# Autodesk Inventor assembly: Assembly12
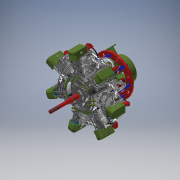
[picture p0: Inventor's stored thumbnail of the model, 180x180]
Saved by Autodesk Inventor 2018 (Build 220112000, 112)
## iProperties
Created: 2023-05-03
Part Number: Assembly12
Document SubType Name: Assembly
Designer: Habib Mohamed
Author: Habib Mohamed
## Documents named in this file (11)
- D:\Inventor\My projects\Rotary Engine\Assembly\Assembly12.iam
- D:\Inventor\My projects\Rotary Engine\Assembly\Assembly10(Suction houe sub assembly).iam
- D:\Inventor\My projects\Rotary Engine\Assembly\Assembly9 (Crank Case Sub Assembly).iam
- D:\Inventor\My projects\Rotary Engine\Component 9 (Suspension Spacer).ipt
- D:\Inventor\My projects\Rotary Engine\Component 10(Assembly Ring).ipt
- D:\Inventor\My projects\Rotary Engine\Assembly\Assembly2 (Intake Pipe Sub Assembly).iam
- C:\Users\Habib Mohamed\Downloads\Exhaust Pipe Sub-Assembly.iam
- D:\Inventor\My projects\Rotary Engine\Component 46(Engine Gas Collector).ipt
- C:\Users\Habib Mohamed\Documents\Inventor\Content Center Files\R2018\en-US\ISO 4762(1)\DIN EN ISO 4762 - M3 x 5.ipt
- C:\Users\Habib Mohamed\Documents\Inventor\Content Center Files\R2018\en-US\ISO 4762(1)\DIN EN ISO 4762 - M4 x 10.ipt
- C:\Users\Habib Mohamed\Documents\Inventor\Content Center Files\R2018\en-US\ISO 10511\ISO 10511 - M5.ipt
## Components (67 placed, 10 different names)
1. Assembly10(Suction houe sub assembly):1 [sub-assembly] — Mate:1, Mate:2, Mate:3, Mate:28, Mate:30, Mate:32, Mate:34, Mate:36, Mate:38, Mate:40
2. Assembly9 (Crank Case Sub Assembly):1 [sub-assembly] — Mate:1, Mate:2, Mate:3, Mate:4, Mate:5, Mate:6, Mate:9, Mate:10, Mate:11, Mate:12, Mate:13, Mate:14, Mate:15, Mate:19, Mate:21, Mate:23, Mate:25, Mate:27, Mate:29, Mate:31, Mate:33, Mate:35, Mate:37, Mate:39
3. Component 10(Assembly Ring):1 — Mate:6, Mate:7, Mate:8, Mate:42
4. Component 46(Engine Gas Collector):1 — Mate:15, Mate:16, Mate:17, Mate:18, Mate:43
5. DIN EN ISO 4762 M4 x 10:1 — Mate:27, Mate:28
6. DIN EN ISO 4762 M4 x 10:2 — Mate:29, Mate:30
7. DIN EN ISO 4762 M4 x 10:3 — Mate:31, Mate:32
8. DIN EN ISO 4762 M4 x 10:4 — Mate:33, Mate:34
9. DIN EN ISO 4762 M4 x 10:5 — Mate:35, Mate:36
10. DIN EN ISO 4762 M4 x 10:6 — Mate:37, Mate:38
11. DIN EN ISO 4762 M4 x 10:7 — Mate:39, Mate:40
12. DIN EN ISO 4762 M3 x 5:1 — Mate:19, Mate:20
13. DIN EN ISO 4762 M3 x 5:2 — Mate:21, Mate:22
14. Assembly2 (Intake Pipe Sub Assembly):1 [sub-assembly] — Mate:9, Mate:10, Mate:11, Mate:20, Mate:22
15. Component 9 (Suspension Spacer):1 — Mate:4, Mate:5, Mate:7, Mate:8, Mate:41
16. DIN EN ISO 10511 M5:1 — Mate:41, Mate:42
17. DIN EN ISO 4762 M3 x 5:3 — Mate:23, Mate:24
18. DIN EN ISO 4762 M3 x 5:4 — Mate:25, Mate:26
19. Exhaust Pipe Sub-Assembly:1 [sub-assembly] — Mate:12, Mate:13, Mate:14, Mate:17, Mate:18, Mate:24, Mate:26
20. DIN EN ISO 4762 M3 x 5:5
21. DIN EN ISO 4762 M3 x 5:6
22. Assembly2 (Intake Pipe Sub Assembly):2 [sub-assembly]
23. Component 9 (Suspension Spacer):2
24. DIN EN ISO 10511 M5:2
25. DIN EN ISO 4762 M3 x 5:7
26. DIN EN ISO 4762 M3 x 5:8
27. Exhaust Pipe Sub-Assembly:2 [sub-assembly]
28. DIN EN ISO 4762 M3 x 5:9
29. DIN EN ISO 4762 M3 x 5:10
30. Assembly2 (Intake Pipe Sub Assembly):3 [sub-assembly]
31. Component 9 (Suspension Spacer):3
32. DIN EN ISO 10511 M5:3
33. DIN EN ISO 4762 M3 x 5:11
34. DIN EN ISO 4762 M3 x 5:12
35. Exhaust Pipe Sub-Assembly:3 [sub-assembly]
36. DIN EN ISO 4762 M3 x 5:13
37. DIN EN ISO 4762 M3 x 5:14
38. Assembly2 (Intake Pipe Sub Assembly):4 [sub-assembly]
39. Component 9 (Suspension Spacer):4
40. DIN EN ISO 10511 M5:4
41. DIN EN ISO 4762 M3 x 5:15
42. DIN EN ISO 4762 M3 x 5:16
43. Exhaust Pipe Sub-Assembly:4 [sub-assembly]
44. DIN EN ISO 4762 M3 x 5:17
45. DIN EN ISO 4762 M3 x 5:18
46. Assembly2 (Intake Pipe Sub Assembly):5 [sub-assembly]
47. Component 9 (Suspension Spacer):5
48. DIN EN ISO 10511 M5:5
49. DIN EN ISO 4762 M3 x 5:19
50. DIN EN ISO 4762 M3 x 5:20
51. Exhaust Pipe Sub-Assembly:5 [sub-assembly]
52. DIN EN ISO 4762 M3 x 5:21
53. DIN EN ISO 4762 M3 x 5:22
54. Assembly2 (Intake Pipe Sub Assembly):6 [sub-assembly]
55. Component 9 (Suspension Spacer):6
56. DIN EN ISO 10511 M5:6
57. DIN EN ISO 4762 M3 x 5:23
58. DIN EN ISO 4762 M3 x 5:24
59. Exhaust Pipe Sub-Assembly:6 [sub-assembly]
60. DIN EN ISO 4762 M3 x 5:25
61. DIN EN ISO 4762 M3 x 5:26
62. Assembly2 (Intake Pipe Sub Assembly):7 [sub-assembly]
63. Component 9 (Suspension Spacer):7
64. DIN EN ISO 10511 M5:7
65. DIN EN ISO 4762 M3 x 5:27
66. DIN EN ISO 4762 M3 x 5:28
67. Exhaust Pipe Sub-Assembly:7 [sub-assembly]
## Component patterns: (7 elements, first: DIN EN ISO 4762 M3 x 5:1 + DIN EN ISO 4762 M3 x 5:2 + Assembly2 (Intake Pipe Sub Assembly):1 + Component 9 (Suspension Spacer):1 + DIN EN ISO 10511 M5:1 + DIN EN ISO 4762 M3 x 5:3 + DIN EN ISO 4762 M3 x 5:4 + Exhaust Pipe Sub-Assembly:1)
## Relationships (43: Mate 43)
- Mate:1: Assembly10(Suction houe sub assembly):1 ↔ Assembly9 (Crank Case Sub Assembly):1
- Mate:2: Assembly10(Suction houe sub assembly):1 ↔ Assembly9 (Crank Case Sub Assembly):1
- Mate:3: Assembly10(Suction houe sub assembly):1 ↔ Assembly9 (Crank Case Sub Assembly):1
- Mate:4: Assembly9 (Crank Case Sub Assembly):1 ↔ Component 9 (Suspension Spacer):1
- Mate:5: Assembly9 (Crank Case Sub Assembly):1 ↔ Component 9 (Suspension Spacer):1
- Mate:6: Assembly9 (Crank Case Sub Assembly):1 ↔ Component 10(Assembly Ring):1
- Mate:7: Component 10(Assembly Ring):1 ↔ Component 9 (Suspension Spacer):1
- Mate:8: Component 10(Assembly Ring):1 ↔ Component 9 (Suspension Spacer):1
- Mate:9: Assembly9 (Crank Case Sub Assembly):1 ↔ Assembly2 (Intake Pipe Sub Assembly):1
- Mate:10: Assembly9 (Crank Case Sub Assembly):1 ↔ Assembly2 (Intake Pipe Sub Assembly):1
- Mate:11: Assembly9 (Crank Case Sub Assembly):1 ↔ Assembly2 (Intake Pipe Sub Assembly):1
- Mate:12: Assembly9 (Crank Case Sub Assembly):1 ↔ Exhaust Pipe Sub-Assembly:1
- Mate:13: Assembly9 (Crank Case Sub Assembly):1 ↔ Exhaust Pipe Sub-Assembly:1
- Mate:14: Assembly9 (Crank Case Sub Assembly):1 ↔ Exhaust Pipe Sub-Assembly:1
- Mate:15: Assembly9 (Crank Case Sub Assembly):1 ↔ Component 46(Engine Gas Collector):1
- Mate:16: Component 46(Engine Gas Collector):1
- Mate:17: Component 46(Engine Gas Collector):1 ↔ Exhaust Pipe Sub-Assembly:1
- Mate:18: Component 46(Engine Gas Collector):1 ↔ Exhaust Pipe Sub-Assembly:1
- Mate:19: Assembly9 (Crank Case Sub Assembly):1 ↔ DIN EN ISO 4762 M3 x 5:1
- Mate:20: DIN EN ISO 4762 M3 x 5:1 ↔ Assembly2 (Intake Pipe Sub Assembly):1
- Mate:21: Assembly9 (Crank Case Sub Assembly):1 ↔ DIN EN ISO 4762 M3 x 5:2
- Mate:22: DIN EN ISO 4762 M3 x 5:2 ↔ Assembly2 (Intake Pipe Sub Assembly):1
- Mate:23: Assembly9 (Crank Case Sub Assembly):1 ↔ DIN EN ISO 4762 M3 x 5:3
- Mate:24: DIN EN ISO 4762 M3 x 5:3 ↔ Exhaust Pipe Sub-Assembly:1
- Mate:25: Assembly9 (Crank Case Sub Assembly):1 ↔ DIN EN ISO 4762 M3 x 5:4
- Mate:26: DIN EN ISO 4762 M3 x 5:4 ↔ Exhaust Pipe Sub-Assembly:1
- Mate:27: Assembly9 (Crank Case Sub Assembly):1 ↔ DIN EN ISO 4762 M4 x 10:1
- Mate:28: Assembly10(Suction houe sub assembly):1 ↔ DIN EN ISO 4762 M4 x 10:1
- Mate:29: Assembly9 (Crank Case Sub Assembly):1 ↔ DIN EN ISO 4762 M4 x 10:2
- Mate:30: Assembly10(Suction houe sub assembly):1 ↔ DIN EN ISO 4762 M4 x 10:2
- Mate:31: Assembly9 (Crank Case Sub Assembly):1 ↔ DIN EN ISO 4762 M4 x 10:3
- Mate:32: Assembly10(Suction houe sub assembly):1 ↔ DIN EN ISO 4762 M4 x 10:3
- Mate:33: Assembly9 (Crank Case Sub Assembly):1 ↔ DIN EN ISO 4762 M4 x 10:4
- Mate:34: Assembly10(Suction houe sub assembly):1 ↔ DIN EN ISO 4762 M4 x 10:4
- Mate:35: Assembly9 (Crank Case Sub Assembly):1 ↔ DIN EN ISO 4762 M4 x 10:5
- Mate:36: Assembly10(Suction houe sub assembly):1 ↔ DIN EN ISO 4762 M4 x 10:5
- Mate:37: Assembly9 (Crank Case Sub Assembly):1 ↔ DIN EN ISO 4762 M4 x 10:6
- Mate:38: Assembly10(Suction houe sub assembly):1 ↔ DIN EN ISO 4762 M4 x 10:6
- Mate:39: Assembly9 (Crank Case Sub Assembly):1 ↔ DIN EN ISO 4762 M4 x 10:7
- Mate:40: Assembly10(Suction houe sub assembly):1 ↔ DIN EN ISO 4762 M4 x 10:7
- Mate:41: Component 9 (Suspension Spacer):1 ↔ DIN EN ISO 10511 M5:1
- Mate:42: Component 10(Assembly Ring):1 ↔ DIN EN ISO 10511 M5:1
- Mate:43: Component 46(Engine Gas Collector):1
